# Autodesk Inventor assembly: composter
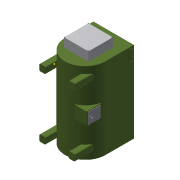
[picture p0: Inventor's stored thumbnail of the model, 180x180]
Saved by Autodesk Inventor 2019 (Build 230136000, 136)
## iProperties
Created: 2020-02-29
Part Number: composter
Document SubType Name: Assembly
Designer: stef_
Author: stef_
## Documents named in this file (9)
- C:\Users\stef_\Documents\Academiejaar 2019-2020\Semester 2\4-Composter\composter.iam
- C:\Users\stef_\Documents\Academiejaar 2019-2020\Semester 1\5-Besturingstechnieken\bak zelf.ipt
- C:\Users\stef_\Documents\Academiejaar 2019-2020\Semester 1\5-Besturingstechnieken\deksel.ipt
- C:\Users\stef_\Documents\Academiejaar 2019-2020\Semester 1\5-Besturingstechnieken\klep.ipt
- C:\Users\stef_\Documents\Academiejaar 2019-2020\Semester 2\4-Composter\aanstuurkast.ipt
- C:\Users\stef_\Documents\Academiejaar 2019-2020\Semester 2\4-Composter\aanstuurkast kap.ipt
- C:\Users\stef_\Documents\Inventor\Content Center Files\R2019\en-US\DIN 125-2  A\DIN 125-2 - B 6,4A.ipt
- C:\Users\stef_\Documents\Inventor\Content Center Files\R2019\en-US\DIN EN ISO 4017\DIN EN ISO 4017 - M6 x 12.ipt
- C:\Users\stef_\Documents\Academiejaar 2019-2020\Semester 2\4-Composter\klep uitlaat.ipt
## Components (16 placed, 8 different names)
1. bak zelf:1 — Flush:1, Flush:3, Mate:1, Flush:5, Flush:7
2. deksel:1 — Mate:1, Flush:4
3. klep:1 — Flush:4
4. aanstuurkast:1 — Flush:5, Flush:6
5. aanstuurkast kap:1 — Flush:6, Mate:2, Mate:3, Mate:4, Mate:5, Mate:6, Mate:7, Mate:8, Mate:9, Insert:3, Insert:4, Insert:5, Insert:6
6. klep uitlaat:1 — Flush:7
7. DIN 125-2 A B 6,4:1 — Mate:2, Mate:3, Insert:1
8. DIN 125-2 A B 6,4:2 — Mate:4, Mate:5
9. DIN 125-2 A B 6,4:3 — Mate:6, Mate:7, Insert:2
10. DIN 125-2 A B 6,4:4 — Mate:8, Mate:9
11. DIN EN ISO 4017 M6 x 12:1 — Insert:1
12. DIN EN ISO 4017 M6 x 12:2 — Insert:2
13. DIN EN ISO 4017 M6 x 12:3 — Insert:3
14. DIN EN ISO 4017 M6 x 12:4 — Insert:4
15. DIN EN ISO 4017 M6 x 12:5 — Insert:5
16. DIN EN ISO 4017 M6 x 12:6 — Insert:6
## Relationships (22: Mate 9, Flush 7, Insert 6)
- Flush:1 (-350 mm): bak zelf:1
- Flush:2 (-344.75 mm)
- Flush:3: bak zelf:1
- Mate:1: bak zelf:1 ↔ deksel:1
- Flush:4: deksel:1 ↔ klep:1
- Flush:5: bak zelf:1 ↔ aanstuurkast:1
- Flush:6: aanstuurkast:1 ↔ aanstuurkast kap:1
- Mate:2: aanstuurkast kap:1 ↔ DIN 125-2 A B 6,4:1
- Mate:3: aanstuurkast kap:1 ↔ DIN 125-2 A B 6,4:1
- Mate:4: aanstuurkast kap:1 ↔ DIN 125-2 A B 6,4:2
- Mate:5: aanstuurkast kap:1 ↔ DIN 125-2 A B 6,4:2
- Mate:6: aanstuurkast kap:1 ↔ DIN 125-2 A B 6,4:3
- Mate:7: aanstuurkast kap:1 ↔ DIN 125-2 A B 6,4:3
- Mate:8: aanstuurkast kap:1 ↔ DIN 125-2 A B 6,4:4
- Mate:9: aanstuurkast kap:1 ↔ DIN 125-2 A B 6,4:4
- Insert:1: DIN 125-2 A B 6,4:1 ↔ DIN EN ISO 4017 M6 x 12:1
- Insert:2: DIN 125-2 A B 6,4:3 ↔ DIN EN ISO 4017 M6 x 12:2
- Insert:3: aanstuurkast kap:1 ↔ DIN EN ISO 4017 M6 x 12:3
- Insert:4: aanstuurkast kap:1 ↔ DIN EN ISO 4017 M6 x 12:4
- Insert:5: aanstuurkast kap:1 ↔ DIN EN ISO 4017 M6 x 12:5
- Insert:6: aanstuurkast kap:1 ↔ DIN EN ISO 4017 M6 x 12:6
- Flush:7: bak zelf:1 ↔ klep uitlaat:1
